# Autodesk Inventor assembly: Roller-ver1-1111-2021
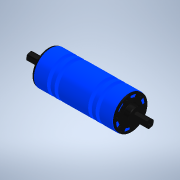
[picture p0: Inventor's stored thumbnail of the model, 180x180]
Saved by Autodesk Inventor 2020 (Build 240168000, 168)
## iProperties
Created: 2021-01-26
Part Number: Roller-ver1-1111-2021
Document SubType Name: Assembly
Designer: Caitlin
Author: Caitlin
## Documents named in this file (4)
- D:\PHRC CADD 2021\PHRC CADD\2020 Infinite Recharge\2021 Infinite Recharge\Chassis\Roller-ver1-1111-2021.iam
- D:\PHRC CADD 2021\PHRC CADD\2020 Infinite Recharge\Storage\Parts\Roller-ver3-1111-2019.ipt
- D:\PHRC CADD 2021\PHRC CADD\Resources\VEXpro Resources\Versa Motion\VersaHub(0.5inHex)-1111-2016.ipt
- D:\PHRC CADD 2021\PHRC CADD\Resources\VEXpro Resources\Shafts\0.5inThunderHexShaft(8in(modified))-1111-2016.ipt
## Components (4 placed, 3 different names)
1. Roller-ver3-1111-2019:1 — Cylindrical:2, Mate:4, Cylindrical:4, Mate:5, Flush:1
2. VersaHub(0.5inHex)-1111-2016:1 — Cylindrical:2, Mate:4, Cylindrical:3, Angle:1
3. 0.5inThunderHexShaft(8in(modified))-1111-2016:1 — Cylindrical:3, Angle:1, Angle:2, Flush:1
4. VersaHub(0.5inHex)-1111-2016:2 — Cylindrical:4, Angle:2, Mate:5
## Relationships (8: CylindricalJoint 3, Mate 2, Angle 2, Flush 1)
- Cylindrical:2: Roller-ver3-1111-2019:1 ↔ VersaHub(0.5inHex)-1111-2016:1
- Mate:4: Roller-ver3-1111-2019:1 ↔ VersaHub(0.5inHex)-1111-2016:1
- Cylindrical:3: VersaHub(0.5inHex)-1111-2016:1 ↔ 0.5inThunderHexShaft(8in(modified))-1111-2016:1
- Angle:1 (0 deg): VersaHub(0.5inHex)-1111-2016:1 ↔ 0.5inThunderHexShaft(8in(modified))-1111-2016:1
- Cylindrical:4: Roller-ver3-1111-2019:1 ↔ VersaHub(0.5inHex)-1111-2016:2
- Angle:2 (0 deg): 0.5inThunderHexShaft(8in(modified))-1111-2016:1 ↔ VersaHub(0.5inHex)-1111-2016:2
- Mate:5: Roller-ver3-1111-2019:1 ↔ VersaHub(0.5inHex)-1111-2016:2
- Flush:1 (-34.925 mm): Roller-ver3-1111-2019:1 ↔ 0.5inThunderHexShaft(8in(modified))-1111-2016:1
